# Autodesk Inventor assembly: 203
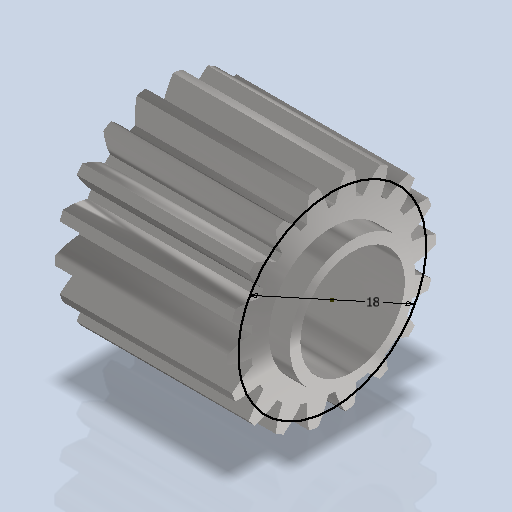
[picture p0: Inventor's stored thumbnail of the model, 512x512]
Saved by Autodesk Inventor 2024 (Build 280153000, 153)
## iProperties
Created: 2024-07-12
Part Number: 203
Document SubType Name: Assembly
Designer: ffogue
Author: ffogue
## Documents named in this file (3)
- C:\Users\ffogue\OneDrive - MuM - OM\Dokumente\Inventor\GearBox\203.iam
- C:\Users\ffogue\OneDrive - MuM - OM\Dokumente\Inventor\GearBox\203 gear.iam
- C:\Users\ffogue\OneDrive - MuM - OM\Dokumente\Inventor\GearBox\203_welle.ipt
## Components (2 placed, 2 different names)
1. 203 gear:1 [sub-assembly] — Einfügen:1
2. 203_welle:1 — Einfügen:1
## Relationships (1: Insert 1)
- Einfügen:1 [Insert] (-16.5 mm): 203 gear:1 ↔ 203_welle:1
